# Autodesk Inventor assembly: y_axis
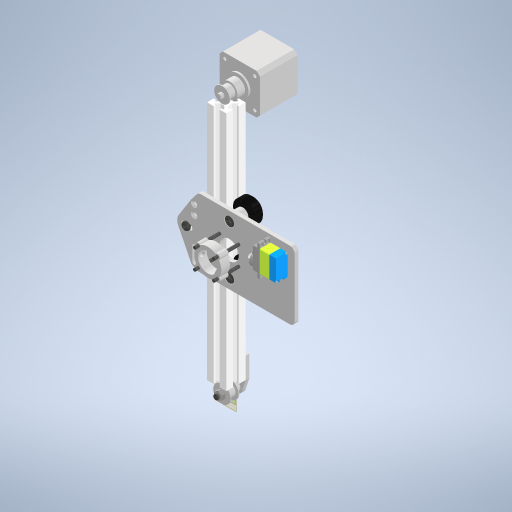
[picture p0: Inventor's stored thumbnail of the model, 512x512]
Saved by Autodesk Inventor 2024 (Build 280153000, 153)
## iProperties
Created: 2026-02-05
Part Number: y_axis
Document SubType Name: Assembly
Designer: SEMEN
Author: SEMEN
## Documents named in this file (19)
- C:\Users\SEMEN\Documents\ETZ2.0\y_axis.iam
- C:\Users\SEMEN\Documents\ETZ2.0\Alumunium T Profile 20x20, 100cm v3.ipt
- C:\Users\SEMEN\Documents\ETZ2.0\motor_x.ipt
- C:\Users\SEMEN\Documents\ETZ2.0\belt_gear_1.ipt
- C:\Users\SEMEN\Documents\ETZ2.0\belt_gear_2.ipt
- C:\Users\SEMEN\Documents\ETZ2.0\belt_tentioner_plane.ipt
- C:\Users\SEMEN\Documents\ETZ2.0\belt_tentioner_washer.ipt
- C:\Users\SEMEN\Documents\Inventor\Content Center Files\R2024\en-US\ISO 7046-1 H(1)\ISO 7046-1 - M5 x 25_ - 4.8 - H - ISO.ipt
- C:\Users\SEMEN\Documents\Inventor\Content Center Files\R2024\en-US\ISO 4032(2)\ISO 4032 - M5 - ISO.ipt
- C:\Users\SEMEN\Documents\Inventor\Content Center Files\R2024\en-US\ISO 7046-1 H(1)\ISO 7046-1 - M4 x 8_ - 4.8 - H - ISO.ipt
- C:\Users\SEMEN\Documents\ETZ2.0\profile_bearing.ipt
- C:\Users\SEMEN\Documents\ETZ2.0\plate_3.ipt
- C:\Users\SEMEN\Documents\Inventor\Content Center Files\R2024\en-US\ISO 7046-1 H(1)\ISO 7046-1 - M3 x 30_ - 4.8 - H - ISO.ipt
- C:\Users\SEMEN\Documents\Inventor\Content Center Files\R2024\en-US\ISO 7046-1 H(1)\ISO 7046-1 - M5 x 30_ - 4.8 - H - ISO.ipt
- C:\Users\SEMEN\Documents\Inventor\Content Center Files\R2024\en-US\ISO 7045  H\ISO 7045 - M4 x 30_ - 4.8 - H - ISO.ipt
- C:\Users\SEMEN\Documents\Inventor\Content Center Files\R2024\en-US\ISO 4032(2)\ISO 4032 - M4 - ISO.ipt
- C:\Users\SEMEN\Documents\ETZ2.0\plate_3_washers.ipt
- C:\Users\SEMEN\Documents\ETZ2.0\marker_holder.ipt
- C:\Users\SEMEN\Documents\ETZ2.0\SG90_Servo_Motor.ipt
## Components (29 placed, 18 different names)
1. motor_y:1 — Mate:1, Mate:2, Angle:1
2. Alumunium T Profile 20x20, 100cm v3:1 — Tangent:1, Flush:1, Mate:2, Angle:1, Tangent:2, Flush:2, Tangent:3, Tangent:4, Flush:3, Flush:4, Tangent:5, Mate:8, Mate:9, Tangent:6, Tangent:7, Mate:10, Mate:14
3. belt_gear_1:1 — Mate:1, Tangent:1, Flush:1, Tangent:2
4. belt_gear_2:1 — Flush:2, Tangent:3, Tangent:4, Mate:5
5. belt_tentioner_plane:1 — Flush:3, Flush:4, Flush:5, Mate:3, Mate:4, Mate:6, Mate:7
6. belt_tentioner_washer:1 — Flush:5
7. profile_bearing:1 — Tangent:5, Mate:8, Mate:11, Mate:12, Mate:21, Mate:24, Mate:29
8. profile_bearing:2 — Mate:9, Tangent:6, Mate:12, Mate:13, Mate:26, Mate:31
9. profile_bearing:3 — Tangent:7, Mate:10, Mate:11, Mate:13, Mate:28
10. plate_3:1 — Mate:14, Mate:15, Mate:16, Mate:17, Mate:18, Mate:19, Mate:20, Mate:22, Mate:33, Mate:34
11. plate_3_washers:1 — Mate:29
12. plate_3_washers:3 — Mate:32, Mate:33
13. plate_3_washers:2 — Mate:30, Mate:31
14. ISO 7046-1 H M5 x 25 - 4.8 - H:1 — Mate:3
15. ISO 4032 M5:1 — Mate:4, Mate:5
16. ISO 7046-1 H M4 x 8 - 4.8 - H:1 — Mate:6
17. ISO 7046-1 H M4 x 8 - 4.8 - H:2 — Mate:7
18. ISO 7046-1 H M3 x 30 - 4.8 - H:1 — Mate:15
19. ISO 7046-1 H M3 x 30 - 4.8 - H:2 — Mate:16
20. ISO 7046-1 H M3 x 30 - 4.8 - H:3 — Mate:17
21. ISO 7046-1 H M3 x 30 - 4.8 - H:4 — Mate:18
22. ISO 7046-1 H M5 x 30 - 4.8 - H:1 — Mate:19, Mate:27, Mate:32
23. ISO 7046-1 H M5 x 30 - 4.8 - H:2 — Mate:20, Mate:25, Mate:30
24. ISO 7045 H M4 x 30 - 4.8 - H:1 — Mate:21, Mate:22, Mate:23
25. ISO 4032 M4:1 — Mate:23, Mate:24
26. ISO 4032 M5:2 — Mate:25, Mate:26
27. ISO 4032 M5:3 — Mate:27, Mate:28
28. marker_holder:1
29. SG90_Servo_Motor:1 — Mate:34
## Relationships (47: Mate 34, Tangent 7, Flush 5, Angle 1)
- Mate:1: motor_y:1 ↔ belt_gear_1:1
- Tangent:1 (1 mm): Alumunium T Profile 20x20, 100cm v3:1 ↔ belt_gear_1:1
- Flush:1 (0.5 mm): Alumunium T Profile 20x20, 100cm v3:1 ↔ belt_gear_1:1
- Mate:2 (4 mm): motor_y:1 ↔ Alumunium T Profile 20x20, 100cm v3:1
- Angle:1 (0 deg): motor_y:1 ↔ Alumunium T Profile 20x20, 100cm v3:1
- Tangent:2 (2 mm): Alumunium T Profile 20x20, 100cm v3:1 ↔ belt_gear_1:1
- Flush:2 (0.7 mm): Alumunium T Profile 20x20, 100cm v3:1 ↔ belt_gear_2:1
- Tangent:3 (1 mm): Alumunium T Profile 20x20, 100cm v3:1 ↔ belt_gear_2:1
- Tangent:4 (1 mm): Alumunium T Profile 20x20, 100cm v3:1 ↔ belt_gear_2:1
- Flush:3: Alumunium T Profile 20x20, 100cm v3:1 ↔ belt_tentioner_plane:1
- Flush:4: Alumunium T Profile 20x20, 100cm v3:1 ↔ belt_tentioner_plane:1
- Flush:5: belt_tentioner_plane:1 ↔ belt_tentioner_washer:1
- Mate:3: belt_tentioner_plane:1 ↔ ISO 7046-1 H M5 x 25 - 4.8 - H:1
- Mate:4: belt_tentioner_plane:1 ↔ ISO 4032 M5:1
- Mate:5: belt_gear_2:1 ↔ ISO 4032 M5:1
- Mate:6: belt_tentioner_plane:1 ↔ ISO 7046-1 H M4 x 8 - 4.8 - H:1
- Mate:7: belt_tentioner_plane:1 ↔ ISO 7046-1 H M4 x 8 - 4.8 - H:2
- Tangent:5: Alumunium T Profile 20x20, 100cm v3:1 ↔ profile_bearing:1
- Mate:8 (-2 mm): Alumunium T Profile 20x20, 100cm v3:1 ↔ profile_bearing:1
- Mate:9 (-2 mm): Alumunium T Profile 20x20, 100cm v3:1 ↔ profile_bearing:2
- Tangent:6: Alumunium T Profile 20x20, 100cm v3:1 ↔ profile_bearing:2
- Tangent:7: Alumunium T Profile 20x20, 100cm v3:1 ↔ profile_bearing:3
- Mate:10 (-2 mm): Alumunium T Profile 20x20, 100cm v3:1 ↔ profile_bearing:3
- Mate:11 (50.8068 mm): profile_bearing:1 ↔ profile_bearing:3
- Mate:12 (50.8068 mm): profile_bearing:1 ↔ profile_bearing:2
- Mate:13 (50.8068 mm): profile_bearing:2 ↔ profile_bearing:3
- Mate:14 (5 mm): Alumunium T Profile 20x20, 100cm v3:1 ↔ plate_3:1
- Mate:15: plate_3:1 ↔ ISO 7046-1 H M3 x 30 - 4.8 - H:1
- Mate:16: plate_3:1 ↔ ISO 7046-1 H M3 x 30 - 4.8 - H:2
- Mate:17: plate_3:1 ↔ ISO 7046-1 H M3 x 30 - 4.8 - H:3
- Mate:18: plate_3:1 ↔ ISO 7046-1 H M3 x 30 - 4.8 - H:4
- Mate:19: plate_3:1 ↔ ISO 7046-1 H M5 x 30 - 4.8 - H:1
- Mate:20: plate_3:1 ↔ ISO 7046-1 H M5 x 30 - 4.8 - H:2
- Mate:21: profile_bearing:1 ↔ ISO 7045 H M4 x 30 - 4.8 - H:1
- Mate:22: plate_3:1 ↔ ISO 7045 H M4 x 30 - 4.8 - H:1
- Mate:23: ISO 7045 H M4 x 30 - 4.8 - H:1 ↔ ISO 4032 M4:1
- Mate:24: profile_bearing:1 ↔ ISO 4032 M4:1
- Mate:25: ISO 7046-1 H M5 x 30 - 4.8 - H:2 ↔ ISO 4032 M5:2
- Mate:26: profile_bearing:2 ↔ ISO 4032 M5:2
- Mate:27: ISO 7046-1 H M5 x 30 - 4.8 - H:1 ↔ ISO 4032 M5:3
- Mate:28: profile_bearing:3 ↔ ISO 4032 M5:3
- Mate:29: profile_bearing:1 ↔ plate_3_washers:1
- Mate:30: plate_3_washers:2 ↔ ISO 7046-1 H M5 x 30 - 4.8 - H:2
- Mate:31: profile_bearing:2 ↔ plate_3_washers:2
- Mate:32: plate_3_washers:3 ↔ ISO 7046-1 H M5 x 30 - 4.8 - H:1
- Mate:33: plate_3:1 ↔ plate_3_washers:3
- Mate:34: plate_3:1 ↔ SG90_Servo_Motor:1
